# Autodesk Inventor assembly: sborka
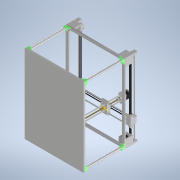
[picture p0: Inventor's stored thumbnail of the model, 180x180]
Saved by Autodesk Inventor 2021 (Build 250183000, 183)
## iProperties
Created: 2023-01-13
Part Number: sborka
Document SubType Name: Assembly
Designer: ignat
Author: ignat
## Documents named in this file (28)
- D:\YandexDisk\2022-2023\Предпроф олимпиада\очный тур\шахматы\inventor\sborka.iam
- D:\YandexDisk\2022-2023\Предпроф олимпиада\очный тур\шахматы\inventor\base_plate.ipt
- D:\YandexDisk\2022-2023\Предпроф олимпиада\очный тур\шахматы\inventor\base_plate_corner_holder.ipt
- D:\YandexDisk\2022-2023\Предпроф олимпиада\очный тур\шахматы\inventor\tube_16_400.ipt
- D:\YandexDisk\2022-2023\Предпроф олимпиада\очный тур\шахматы\inventor\top_plate.ipt
- D:\YandexDisk\2022-2023\Предпроф олимпиада\очный тур\шахматы\inventor\motor_holder.ipt
- D:\YandexDisk\2022-2023\Предпроф олимпиада\очный тур\шахматы\inventor\motor_holder_mirror.ipt
- D:\YandexDisk\2022-2023\Предпроф олимпиада\очный тур\шахматы\inventor\bearing_holder.ipt
- D:\YandexDisk\2022-2023\Предпроф олимпиада\очный тур\шахматы\inventor\bearing_holder_mirror.ipt
- D:\YandexDisk\2022-2023\Предпроф олимпиада\очный тур\шахматы\inventor\rail_450.ipt
- D:\YandexDisk\2022-2023\Предпроф олимпиада\очный тур\шахматы\inventor\Nema17.ipt
- D:\YandexDisk\2022-2023\Предпроф олимпиада\очный тур\шахматы\inventor\625zz.ipt
- D:\YandexDisk\2022-2023\Предпроф олимпиада\очный тур\шахматы\inventor\GT2-20t.ipt
- D:\YandexDisk\2022-2023\Предпроф олимпиада\очный тур\шахматы\inventor\x_rail_holder.ipt
- D:\YandexDisk\2022-2023\Предпроф олимпиада\очный тур\шахматы\inventor\LM8LUU.ipt
- D:\YandexDisk\2022-2023\Предпроф олимпиада\очный тур\шахматы\inventor\rail_381.ipt
- D:\YandexDisk\2022-2023\Предпроф олимпиада\очный тур\шахматы\inventor\LM8SUU.ipt
- D:\YandexDisk\2022-2023\Предпроф олимпиада\очный тур\шахматы\inventor\x_slider.ipt
- D:\YandexDisk\2022-2023\Предпроф олимпиада\очный тур\шахматы\inventor\LM8UU.ipt
- D:\YandexDisk\2022-2023\Предпроф олимпиада\очный тур\шахматы\inventor\M8_nut.ipt
- D:\YandexDisk\2022-2023\Предпроф олимпиада\очный тур\шахматы\inventor\gt2_belt.ipt
- D:\YandexDisk\2022-2023\Предпроф олимпиада\очный тур\шахматы\inventor\rail_300.ipt
- D:\YandexDisk\2022-2023\Предпроф олимпиада\очный тур\шахматы\inventor\z_slider_bearing_holder.ipt
- D:\YandexDisk\2022-2023\Предпроф олимпиада\очный тур\шахматы\inventor\z_slider_motor_holder.ipt
- D:\YandexDisk\2022-2023\Предпроф олимпиада\очный тур\шахматы\inventor\mufta_5x8.ipt
- D:\YandexDisk\2022-2023\Предпроф олимпиада\очный тур\шахматы\inventor\T8_vint.ipt
- D:\YandexDisk\2022-2023\Предпроф олимпиада\очный тур\шахматы\inventor\prostavka_6,6.ipt
- D:\YandexDisk\2022-2023\Предпроф олимпиада\очный тур\шахматы\inventor\prostavka_7,6.ipt
## Components (77 placed, 27 different names)
1. base_plate:1 — Совмещение:1, Совмещение:2, Совмещение:3, Совмещение:4, Заподлицо:1, Заподлицо:2, Заподлицо:3, Заподлицо:4, Заподлицо:5, Заподлицо:6, Заподлицо:7, Заподлицо:8, Совмещение:28, Совмещение:29
2. base_plate_corner_holder:1 — Совмещение:1, Заподлицо:7, Заподлицо:8, Вставка:3, Заподлицо:9
3. base_plate_corner_holder:2 — Совмещение:2, Заподлицо:5, Заподлицо:6, Вставка:4, Заподлицо:10
4. base_plate_corner_holder:3 — Совмещение:3, Заподлицо:3, Заподлицо:4, Вставка:2, Заподлицо:12
5. base_plate_corner_holder:4 — Совмещение:4, Заподлицо:1, Заподлицо:2, Вставка:1, Заподлицо:11
6. tube_16_400:1 — Вставка:1, Вставка:5
7. tube_16_400:2 — Вставка:2, Вставка:6
8. tube_16_400:3 — Вставка:4, Вставка:7
9. tube_16_400:4 — Вставка:3, Вставка:8
10. base_plate_corner_holder:5 — Вставка:5, Заподлицо:11, Заподлицо:19, Заподлицо:20
11. base_plate_corner_holder:6 — Вставка:6, Заподлицо:12, Вставка:10, Заподлицо:21, Заподлицо:22
12. base_plate_corner_holder:7 — Вставка:7, Заподлицо:10, Вставка:9, Заподлицо:15, Заподлицо:16
13. base_plate_corner_holder:8 — Вставка:8, Заподлицо:9, Заподлицо:17, Заподлицо:18
14. top_plate:1 — Вставка:9, Вставка:10, Совмещение:5, Заподлицо:13, Заподлицо:14
15. top_plate:2 — Совмещение:5, Заподлицо:13, Заподлицо:14, Совмещение:6, Совмещение:7, Совмещение:8, Совмещение:9
16. motor_holder:1 — Совмещение:6, Заподлицо:15, Заподлицо:16, Вставка:13, Вставка:16
17. motor_holder_mirror:1 — Совмещение:7, Заподлицо:17, Заподлицо:18, Вставка:14, Вставка:15
18. bearing_holder:1 — Совмещение:9, Заподлицо:21, Заподлицо:22, Вставка:11, Вставка:18, Вставка:20, Совмещение:10
19. bearing_holder_mirror:1 — Совмещение:8, Заподлицо:19, Заподлицо:20, Вставка:12, Вставка:17, Вставка:19, Совмещение:11
20. rail_450:1 — Вставка:11, Совмещение:12
21. rail_450:2 — Вставка:12, Совмещение:17
22. Nema17:1 — Вставка:13, Вставка:16, Вставка:22
23. Nema17:2 — Вставка:14, Вставка:15, Вставка:21
24. 625zz:1 — Вставка:20, Вставка:64
25. 625zz:2 — Вставка:19, Вставка:66
26. 625zz:3 — Вставка:18, Вставка:65
27. 625zz:4 — Вставка:17, Вставка:67
28. GT2-20t:1 — Совмещение:11, Заподлицо:23
29. GT2-20t:2 — Совмещение:10, Заподлицо:24
30. GT2-20t:3 — Вставка:22, Заподлицо:23, Заподлицо:28, Заподлицо:29, Совмещение:22
31. GT2-20t:4 — Вставка:21, Заподлицо:24, Заподлицо:25, Заподлицо:26, Совмещение:21, Совмещение:23
32. x_rail_holder:1 — Вставка:23, Совмещение:13, Совмещение:14, Вставка:24, Вставка:25, Вставка:26, Вставка:27, Заподлицо:27, Вставка:53, Вставка:54
33. LM8LUU:1 — Совмещение:12, Вставка:23
34. GT2-20t:5 — Совмещение:13, Заподлицо:26, Совмещение:24
35. GT2-20t:6 — Совмещение:14, Заподлицо:25
36. 625zz:5 — Вставка:27, Вставка:61
37. 625zz:6 — Вставка:26, Вставка:60
38. 625zz:7 — Вставка:25, Вставка:62
39. 625zz:8 — Вставка:24, Вставка:63
40. x_rail_holder:2 — Заподлицо:27, Вставка:52, Вставка:55
41. LM8LUU:2 — Совмещение:17
42. GT2-20t:7 — Заподлицо:28
43. GT2-20t:8 — Заподлицо:29
44. 625zz:9 — Вставка:58
45. 625zz:10 — Вставка:57
46. 625zz:11 — Вставка:59
47. 625zz:12 — Вставка:56
48. rail_381:1 — Совмещение:18, Вставка:54, Вставка:55
49. rail_381:2 — Совмещение:19, Вставка:52, Вставка:53
50. LM8SUU:1 — Вставка:40
51. x_slider:1 — Вставка:37, Вставка:38, Вставка:39, Вставка:40, Вставка:41, Вставка:42, Вставка:43, Совмещение:20, Совмещение:27
52. LM8SUU:2 — Вставка:39
53. LM8SUU:3 — Вставка:38, Совмещение:19
54. LM8SUU:4 — Вставка:37, Совмещение:18
55. LM8UU:1 — Вставка:42, Совмещение:25
56. M8_nut:1 — Вставка:43, Совмещение:20
57. LM8UU:2 — Вставка:41, Совмещение:26
58. gt2_belt:1 — Совмещение:21, Совмещение:22, Совмещение:23, Совмещение:24
59. rail_300:1 — Вставка:45, Вставка:47, Совмещение:26
60. z_slider_bearing_holder:1 — Вставка:44, Вставка:45
61. z_slider_motor_holder:1 — Вставка:46, Вставка:47, Совмещение:27, Вставка:48, Вставка:49
62. rail_300:2 — Вставка:44, Вставка:46, Совмещение:25
63. Nema17:3 — Вставка:48, Вставка:49, Вставка:50
64. mufta_5x8:1 — Вставка:50, Вставка:51
65. T8_vint:1 — Вставка:51
66. prostavka_6,6:1 — Вставка:56
67. prostavka_6,6:2 — Вставка:57
68. prostavka_6,6:3 — Вставка:58
69. prostavka_6,6:4 — Вставка:59
70. prostavka_6,6:5 — Вставка:60
71. prostavka_6,6:6 — Вставка:61
72. prostavka_6,6:7 — Вставка:62
73. prostavka_6,6:8 — Вставка:63
74. prostavka_6,6:9 — Вставка:65
75. prostavka_7,6:1 — Вставка:64
76. prostavka_6,6:10 — Вставка:67
77. prostavka_7,6:2 — Вставка:66
## Relationships (121: Insert 63, Mate 29, Flush 29)
- Совмещение:1 [Mate]: base_plate:1 ↔ base_plate_corner_holder:1
- Совмещение:2 [Mate]: base_plate:1 ↔ base_plate_corner_holder:2
- Совмещение:3 [Mate]: base_plate:1 ↔ base_plate_corner_holder:3
- Совмещение:4 [Mate]: base_plate:1 ↔ base_plate_corner_holder:4
- Заподлицо:1 [Flush]: base_plate:1 ↔ base_plate_corner_holder:4
- Заподлицо:2 [Flush]: base_plate:1 ↔ base_plate_corner_holder:4
- Заподлицо:3 [Flush]: base_plate:1 ↔ base_plate_corner_holder:3
- Заподлицо:4 [Flush]: base_plate:1 ↔ base_plate_corner_holder:3
- Заподлицо:5 [Flush]: base_plate:1 ↔ base_plate_corner_holder:2
- Заподлицо:6 [Flush]: base_plate:1 ↔ base_plate_corner_holder:2
- Заподлицо:7 [Flush]: base_plate:1 ↔ base_plate_corner_holder:1
- Заподлицо:8 [Flush]: base_plate:1 ↔ base_plate_corner_holder:1
- Вставка:1 [Insert]: base_plate_corner_holder:4 ↔ tube_16_400:1
- Вставка:2 [Insert]: base_plate_corner_holder:3 ↔ tube_16_400:2
- Вставка:3 [Insert]: base_plate_corner_holder:1 ↔ tube_16_400:4
- Вставка:4 [Insert]: base_plate_corner_holder:2 ↔ tube_16_400:3
- Вставка:5 [Insert]: tube_16_400:1 ↔ base_plate_corner_holder:5
- Вставка:6 [Insert]: tube_16_400:2 ↔ base_plate_corner_holder:6
- Вставка:7 [Insert]: tube_16_400:3 ↔ base_plate_corner_holder:7
- Вставка:8 [Insert]: tube_16_400:4 ↔ base_plate_corner_holder:8
- Заподлицо:9 [Flush]: base_plate_corner_holder:1 ↔ base_plate_corner_holder:8
- Заподлицо:10 [Flush]: base_plate_corner_holder:2 ↔ base_plate_corner_holder:7
- Заподлицо:11 [Flush]: base_plate_corner_holder:4 ↔ base_plate_corner_holder:5
- Заподлицо:12 [Flush]: base_plate_corner_holder:3 ↔ base_plate_corner_holder:6
- Вставка:9 [Insert]: base_plate_corner_holder:7 ↔ top_plate:1
- Вставка:10 [Insert]: base_plate_corner_holder:6 ↔ top_plate:1
- Совмещение:5 [Mate]: top_plate:1 ↔ top_plate:2
- Заподлицо:13 [Flush]: top_plate:1 ↔ top_plate:2
- Заподлицо:14 [Flush]: top_plate:1 ↔ top_plate:2
- Совмещение:6 [Mate]: top_plate:2 ↔ motor_holder:1
- Заподлицо:15 [Flush]: base_plate_corner_holder:7 ↔ motor_holder:1
- Заподлицо:16 [Flush]: base_plate_corner_holder:7 ↔ motor_holder:1
- Совмещение:7 [Mate]: top_plate:2 ↔ motor_holder_mirror:1
- Заподлицо:17 [Flush]: base_plate_corner_holder:8 ↔ motor_holder_mirror:1
- Заподлицо:18 [Flush]: base_plate_corner_holder:8 ↔ motor_holder_mirror:1
- Совмещение:8 [Mate]: top_plate:2 ↔ bearing_holder_mirror:1
- Заподлицо:19 [Flush]: base_plate_corner_holder:5 ↔ bearing_holder_mirror:1
- Заподлицо:20 [Flush]: base_plate_corner_holder:5 ↔ bearing_holder_mirror:1
- Совмещение:9 [Mate]: top_plate:2 ↔ bearing_holder:1
- Заподлицо:21 [Flush]: base_plate_corner_holder:6 ↔ bearing_holder:1
- Заподлицо:22 [Flush]: base_plate_corner_holder:6 ↔ bearing_holder:1
- Вставка:11 [Insert]: bearing_holder:1 ↔ rail_450:1
- Вставка:12 [Insert]: bearing_holder_mirror:1 ↔ rail_450:2
- Вставка:13 [Insert]: motor_holder:1 ↔ Nema17:1
- Вставка:14 [Insert]: motor_holder_mirror:1 ↔ Nema17:2
- Вставка:15 [Insert]: motor_holder_mirror:1 ↔ Nema17:2
- Вставка:16 [Insert]: motor_holder:1 ↔ Nema17:1
- Вставка:17 [Insert]: bearing_holder_mirror:1 ↔ 625zz:4
- Вставка:18 [Insert]: bearing_holder:1 ↔ 625zz:3
- Вставка:19 [Insert]: bearing_holder_mirror:1 ↔ 625zz:2
- Вставка:20 [Insert]: bearing_holder:1 ↔ 625zz:1
- Вставка:21 [Insert] (2 mm): Nema17:2 ↔ GT2-20t:4
- Вставка:22 [Insert] (2 mm): Nema17:1 ↔ GT2-20t:3
- Совмещение:10 [Mate]: bearing_holder:1 ↔ GT2-20t:2
- Совмещение:11 [Mate]: bearing_holder_mirror:1 ↔ GT2-20t:1
- Заподлицо:23 [Flush]: GT2-20t:1 ↔ GT2-20t:3
- Заподлицо:24 [Flush]: GT2-20t:2 ↔ GT2-20t:4
- Совмещение:12 [Mate]: rail_450:1 ↔ LM8LUU:1
- Вставка:23 [Insert]: x_rail_holder:1 ↔ LM8LUU:1
- Совмещение:13 [Mate]: x_rail_holder:1 ↔ GT2-20t:5
- Совмещение:14 [Mate]: x_rail_holder:1 ↔ GT2-20t:6
- Заподлицо:25 [Flush]: GT2-20t:4 ↔ GT2-20t:6
- Заподлицо:26 [Flush]: GT2-20t:4 ↔ GT2-20t:5
- Вставка:24 [Insert]: x_rail_holder:1 ↔ 625zz:8
- Вставка:25 [Insert]: x_rail_holder:1 ↔ 625zz:7
- Вставка:26 [Insert]: x_rail_holder:1 ↔ 625zz:6
- Вставка:27 [Insert]: x_rail_holder:1 ↔ 625zz:5
- [Insert]: x_rail_holder:2 ↔ LM8LUU:2
- [Mate]: x_rail_holder:2 ↔ GT2-20t:7
- [Mate]: x_rail_holder:2 ↔ GT2-20t:8
- [Insert]: x_rail_holder:2 ↔ 625zz:12
- [Insert]: x_rail_holder:2 ↔ 625zz:11
- [Insert]: x_rail_holder:2 ↔ 625zz:10
- [Insert]: x_rail_holder:2 ↔ 625zz:9
- Совмещение:17 [Mate]: rail_450:2 ↔ LM8LUU:2
- Заподлицо:27 [Flush]: x_rail_holder:1 ↔ x_rail_holder:2
- Заподлицо:28 [Flush]: GT2-20t:3 ↔ GT2-20t:7
- Заподлицо:29 [Flush]: GT2-20t:3 ↔ GT2-20t:8
- Вставка:37 [Insert]: x_slider:1 ↔ LM8SUU:4
- Вставка:38 [Insert]: x_slider:1 ↔ LM8SUU:3
- Вставка:39 [Insert]: x_slider:1 ↔ LM8SUU:2
- Вставка:40 [Insert]: LM8SUU:1 ↔ x_slider:1
- Совмещение:18 [Mate]: rail_381:1 ↔ LM8SUU:4
- Совмещение:19 [Mate]: rail_381:2 ↔ LM8SUU:3
- Вставка:41 [Insert]: x_slider:1 ↔ LM8UU:2
- Вставка:42 [Insert]: x_slider:1 ↔ LM8UU:1
- Вставка:43 [Insert]: x_slider:1 ↔ M8_nut:1
- Совмещение:20 [Mate]: x_slider:1 ↔ M8_nut:1
- Совмещение:21 [Mate]: GT2-20t:4 ↔ gt2_belt:1
- Совмещение:22 [Mate]: GT2-20t:3 ↔ gt2_belt:1
- Совмещение:23 [Mate]: GT2-20t:4 ↔ gt2_belt:1
- Совмещение:24 [Mate]: GT2-20t:5 ↔ gt2_belt:1
- Вставка:44 [Insert]: z_slider_bearing_holder:1 ↔ rail_300:2
- Вставка:45 [Insert]: rail_300:1 ↔ z_slider_bearing_holder:1
- Вставка:46 [Insert]: z_slider_motor_holder:1 ↔ rail_300:2
- Вставка:47 [Insert]: rail_300:1 ↔ z_slider_motor_holder:1
- Совмещение:25 [Mate]: LM8UU:1 ↔ rail_300:2
- Совмещение:26 [Mate]: LM8UU:2 ↔ rail_300:1
- Совмещение:27 [Mate] (100 mm): x_slider:1 ↔ z_slider_motor_holder:1
- Вставка:48 [Insert]: z_slider_motor_holder:1 ↔ Nema17:3
- Вставка:49 [Insert]: z_slider_motor_holder:1 ↔ Nema17:3
- Вставка:50 [Insert]: Nema17:3 ↔ mufta_5x8:1
- Вставка:51 [Insert]: mufta_5x8:1 ↔ T8_vint:1
- Совмещение:28 [Mate]: base_plate:1
- Совмещение:29 [Mate]: base_plate:1
- Вставка:52 [Insert]: x_rail_holder:2 ↔ rail_381:2
- Вставка:53 [Insert]: x_rail_holder:1 ↔ rail_381:2
- Вставка:54 [Insert]: x_rail_holder:1 ↔ rail_381:1
- Вставка:55 [Insert]: x_rail_holder:2 ↔ rail_381:1
- Вставка:56 [Insert]: 625zz:12 ↔ prostavka_6,6:1
- Вставка:57 [Insert]: 625zz:10 ↔ prostavka_6,6:2
- Вставка:58 [Insert]: 625zz:9 ↔ prostavka_6,6:3
- Вставка:59 [Insert]: 625zz:11 ↔ prostavka_6,6:4
- Вставка:60 [Insert]: 625zz:6 ↔ prostavka_6,6:5
- Вставка:61 [Insert]: 625zz:5 ↔ prostavka_6,6:6
- Вставка:62 [Insert]: 625zz:7 ↔ prostavka_6,6:7
- Вставка:63 [Insert]: 625zz:8 ↔ prostavka_6,6:8
- Вставка:64 [Insert]: 625zz:1 ↔ prostavka_7,6:1
- Вставка:65 [Insert]: 625zz:3 ↔ prostavka_6,6:9
- Вставка:66 [Insert]: 625zz:2 ↔ prostavka_7,6:2
- Вставка:67 [Insert]: 625zz:4 ↔ prostavka_6,6:10
## Named parameters: d69_d65 = 0 mm, d70_d66 = 0 mm, d71_d67 = 0 mm, d72_d68 = 0 mm, d73_d60 = 0 mm, d74_d61 = 0 mm, d75_d62 = 0 mm
